# Autodesk Inventor assembly: platetest
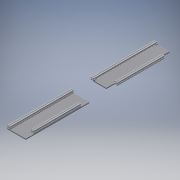
[picture p0: Inventor's stored thumbnail of the model, 180x180]
Saved by Autodesk Inventor 2017 (Build 210142000, 142)
## iProperties
Created: 2018-04-18
Part Number: platetest
Document SubType Name: Assembly
Designer: User
Author: User
## Documents named in this file (4)
- C:\Robotics\CAD\2018-19_CAD\Offseason\platetest.iam
- C:\Robotics\CAD\2018-19_CAD\Offseason\FrameTestOutsidePlate.iam
- C:\Robotics\CAD\2018-19_CAD\Offseason\FrameTestinsidePlate.ipt
- C:\Robotics\CAD\2018-19_CAD\Offseason\platetestoutside.ipt
## Components (4 placed, 3 different names)
1. FrameTestOutsidePlate:1 [sub-assembly] — Flush:1, Flush:2, Flush:5, Mate:3, Flush:6, Mate:4
2. FrameTestinsidePlate:1 — Flush:5, Mate:3, Flush:6
3. FrameTestOutsidePlate:2 [sub-assembly] — Flush:1, Flush:2, Mate:1, Flush:3, Flush:4, Mate:4
4. platetestoutside:1 — Mate:1, Flush:3, Flush:4
## Relationships (9: Flush 6, Mate 3)
- Flush:1: FrameTestOutsidePlate:1 ↔ FrameTestOutsidePlate:2
- Flush:2: FrameTestOutsidePlate:1 ↔ FrameTestOutsidePlate:2
- Mate:1: FrameTestOutsidePlate:2 ↔ platetestoutside:1
- Flush:3: FrameTestOutsidePlate:2 ↔ platetestoutside:1
- Flush:4: FrameTestOutsidePlate:2 ↔ platetestoutside:1
- Flush:5: FrameTestOutsidePlate:1 ↔ FrameTestinsidePlate:1
- Mate:3: FrameTestOutsidePlate:1 ↔ FrameTestinsidePlate:1
- Flush:6: FrameTestOutsidePlate:1 ↔ FrameTestinsidePlate:1
- Mate:4 (254 mm): FrameTestOutsidePlate:1 ↔ FrameTestOutsidePlate:2
